# Autodesk Inventor assembly: BG002_trajan20_22
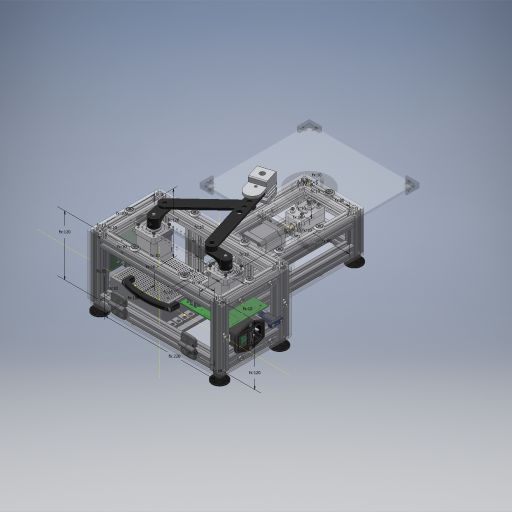
[picture p0: Inventor's stored thumbnail of the model, 512x512]
Saved by Autodesk Inventor 2023 (Build 270158000, 158)
## iProperties
Company: HTBLA Kaindorf
RuleStatus: InUse
Created: 2022-11-06
Part Number: BG002_trajan20_22
Project: Zeichenmaschine_neu
Material: Generisch
Description: Zusammenstellung
Document SubType Name: Assembly
Designer: trajan20
AfterDocNew0: iProperties-Editor_aufrufen
Author: jan
Keywords: 2022
## Documents named in this file (9)
- C:\Users\eligo\Desktop\repo_construction\DrawMachineConstruction\inventor\BG002_trajan20_22_Zeichenmaschine_neu_Zusammenstellung.iam
- C:\Users\eligo\Desktop\repo_construction\DrawMachineConstruction\inventor\BG001_trajan20_22_Zeichenmaschine_neu_Gerüst_mit_Platten.iam
- C:\Users\eligo\Desktop\repo_construction\DrawMachineConstruction\inventor\BG101_trajan20_22_Zeichenmaschine_neu_Gelenke.iam
- C:\Users\eligo\Desktop\repo_construction\DrawMachineConstruction\inventor\BG102_trajan20_22_Zeichenmaschine_neu_Papierplatte.iam
- C:\Users\eligo\Desktop\repo_construction\DrawMachineConstruction\inventor\BG103_trajan20_22_Zeichenmaschine_neu_Stifthalter.iam
- C:\Users\eligo\Desktop\repo_construction\DrawMachineConstruction\inventor\BT301_trajan20_21_Zeichenmaschine_v2_gelenk 1.ipt
- C:\Users\eligo\Desktop\repo_construction\DrawMachineConstruction\inventor\BT301_trajan20_21_Zeichenmaschine_v2_gelenk a.ipt
- C:\Users\eligo\Desktop\repo_construction\DrawMachineConstruction\inventor\BT303_trajan20_21_Zeichenmaschine_v2_gelenk b.ipt
- C:\Users\eligo\Desktop\repo_construction\DrawMachineConstruction\inventor\BT505_trajan20_22_Zeichenmaschine_neu_Stifthalterung_3DDruck.ipt
## Components (9 placed, 8 different names)
1. BG001_trajan20_22_Zeichenmaschine_neu_Gerüst_mit_Platten:1 [sub-assembly] — Passend:4, Passend:5, Passend:6, Passend:7, Passend:8, Passend:24, Passend:25, Passend:26, Passend:27, Winkel:2, Winkel:3
2. BG101_trajan20_22_Zeichenmaschine_neu_Gelenke:1 [sub-assembly] — Passend:4, Passend:5, Passend:6
3. BG102_trajan20_22_Zeichenmaschine_neu_Papierplatte:1 [sub-assembly] — Passend:7, Passend:8, Winkel:3
4. BG103_trajan20_22_Zeichenmaschine_neu_Stifthalter:2 [sub-assembly] — Passend:36, Passend:37, Passend:38
5. BT505_trajan20_22_Zeichenmaschine_neu_Stifthalterung_3DDruck:1 — Passend:40, Passend:41, Passend:42
6. BT301_trajan20_21_Zeichenmaschine_v2_gelenk 1:1 — Passend:24, Passend:25, Passend:31, Passend:32, Winkel:1
7. BT301_trajan20_21_Zeichenmaschine_v2_gelenk 1:2 — Passend:26, Passend:27, Passend:33, Passend:34, Winkel:1, Winkel:2
8. BT301_trajan20_21_Zeichenmaschine_v2_gelenk a:1 — Passend:31, Passend:32, Passend:35
9. BT303_trajan20_21_Zeichenmaschine_v2_gelenk b:1 — Passend:33, Passend:34, Passend:35, Passend:36, Passend:37, Passend:38, Passend:40, Passend:41, Passend:42
## Relationships (23: Mate 20, Angle 3)
- Passend:4 [Mate]: BG001_trajan20_22_Zeichenmaschine_neu_Gerüst_mit_Platten:1 ↔ BG101_trajan20_22_Zeichenmaschine_neu_Gelenke:1
- Passend:5 [Mate] (10 mm): BG001_trajan20_22_Zeichenmaschine_neu_Gerüst_mit_Platten:1 ↔ BG101_trajan20_22_Zeichenmaschine_neu_Gelenke:1
- Passend:6 [Mate]: BG001_trajan20_22_Zeichenmaschine_neu_Gerüst_mit_Platten:1 ↔ BG101_trajan20_22_Zeichenmaschine_neu_Gelenke:1
- Passend:7 [Mate]: BG001_trajan20_22_Zeichenmaschine_neu_Gerüst_mit_Platten:1 ↔ BG102_trajan20_22_Zeichenmaschine_neu_Papierplatte:1
- Passend:8 [Mate] (1 mm): BG001_trajan20_22_Zeichenmaschine_neu_Gerüst_mit_Platten:1 ↔ BG102_trajan20_22_Zeichenmaschine_neu_Papierplatte:1
- Passend:24 [Mate]: BG001_trajan20_22_Zeichenmaschine_neu_Gerüst_mit_Platten:1 ↔ BT301_trajan20_21_Zeichenmaschine_v2_gelenk 1:1
- Passend:25 [Mate]: BG001_trajan20_22_Zeichenmaschine_neu_Gerüst_mit_Platten:1 ↔ BT301_trajan20_21_Zeichenmaschine_v2_gelenk 1:1
- Passend:26 [Mate]: BG001_trajan20_22_Zeichenmaschine_neu_Gerüst_mit_Platten:1 ↔ BT301_trajan20_21_Zeichenmaschine_v2_gelenk 1:2
- Passend:27 [Mate]: BG001_trajan20_22_Zeichenmaschine_neu_Gerüst_mit_Platten:1 ↔ BT301_trajan20_21_Zeichenmaschine_v2_gelenk 1:2
- Passend:31 [Mate]: BT301_trajan20_21_Zeichenmaschine_v2_gelenk 1:1 ↔ BT301_trajan20_21_Zeichenmaschine_v2_gelenk a:1
- Passend:32 [Mate]: BT301_trajan20_21_Zeichenmaschine_v2_gelenk 1:1 ↔ BT301_trajan20_21_Zeichenmaschine_v2_gelenk a:1
- Passend:33 [Mate]: BT301_trajan20_21_Zeichenmaschine_v2_gelenk 1:2 ↔ BT303_trajan20_21_Zeichenmaschine_v2_gelenk b:1
- Passend:34 [Mate]: BT301_trajan20_21_Zeichenmaschine_v2_gelenk 1:2 ↔ BT303_trajan20_21_Zeichenmaschine_v2_gelenk b:1
- Passend:35 [Mate]: BT301_trajan20_21_Zeichenmaschine_v2_gelenk a:1 ↔ BT303_trajan20_21_Zeichenmaschine_v2_gelenk b:1
- Passend:36 [Mate]: BG103_trajan20_22_Zeichenmaschine_neu_Stifthalter:2 ↔ BT303_trajan20_21_Zeichenmaschine_v2_gelenk b:1
- Passend:37 [Mate]: BG103_trajan20_22_Zeichenmaschine_neu_Stifthalter:2 ↔ BT303_trajan20_21_Zeichenmaschine_v2_gelenk b:1
- Passend:38 [Mate]: BG103_trajan20_22_Zeichenmaschine_neu_Stifthalter:2 ↔ BT303_trajan20_21_Zeichenmaschine_v2_gelenk b:1
- Winkel:1 [Angle] (-102 deg): BT301_trajan20_21_Zeichenmaschine_v2_gelenk 1:1 ↔ BT301_trajan20_21_Zeichenmaschine_v2_gelenk 1:2
- Winkel:2 [Angle] (0 deg): BG001_trajan20_22_Zeichenmaschine_neu_Gerüst_mit_Platten:1 ↔ BT301_trajan20_21_Zeichenmaschine_v2_gelenk 1:2
- Winkel:3 [Angle] (0 deg): BG001_trajan20_22_Zeichenmaschine_neu_Gerüst_mit_Platten:1 ↔ BG102_trajan20_22_Zeichenmaschine_neu_Papierplatte:1
- Passend:40 [Mate]: BT505_trajan20_22_Zeichenmaschine_neu_Stifthalterung_3DDruck:1 ↔ BT303_trajan20_21_Zeichenmaschine_v2_gelenk b:1
- Passend:41 [Mate]: BT505_trajan20_22_Zeichenmaschine_neu_Stifthalterung_3DDruck:1 ↔ BT303_trajan20_21_Zeichenmaschine_v2_gelenk b:1
- Passend:42 [Mate]: BT505_trajan20_22_Zeichenmaschine_neu_Stifthalterung_3DDruck:1 ↔ BT303_trajan20_21_Zeichenmaschine_v2_gelenk b:1
